# Autodesk Inventor assembly: kiteAssembly
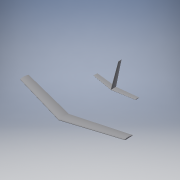
[picture p0: Inventor's stored thumbnail of the model, 180x180]
Saved by Autodesk Inventor 2019.3 (Build 233278000, 278)
## iProperties
Created: 2019-06-24
Part Number: kiteAssembly
Document SubType Name: Assembly
Designer: asiddiq2
Mass: 945352 g
Surface Area: 240754 cm^2
Volume: 945352 cm^3
Density: 1 g/cm^3
Author: asiddiq2
## Documents named in this file (4)
- C:\Users\asiddiq2\Desktop\OCT_project\CAD_models\kiteAssembly.iam
- C:\Users\asiddiq2\Desktop\OCT_project\CAD_models\kite\camberedWing.ipt
- C:\Users\asiddiq2\Desktop\OCT_project\CAD_models\kite\symmetricHS.ipt
- C:\Users\asiddiq2\Desktop\OCT_project\CAD_models\kite\symmetricVS.ipt
## Components (3 placed, 3 different names)
1. camberedWing:1 — Flush:1, Flush:2, Flush:5, Flush:6, Flush:7, Flush:8
2. symmetricHS:1 — Flush:1, Flush:2, Flush:3, Mate:1, Flush:4, Flush:5
3. symmetricVS:1 — Flush:3, Mate:1, Flush:4
## Relationships (9: Flush 8, Mate 1)
- Flush:1: camberedWing:1 ↔ symmetricHS:1
- Flush:2: camberedWing:1 ↔ symmetricHS:1
- Flush:3: symmetricHS:1 ↔ symmetricVS:1
- Mate:1: symmetricHS:1 ↔ symmetricVS:1
- Flush:4: symmetricHS:1 ↔ symmetricVS:1
- Flush:5 (5000 mm): camberedWing:1 ↔ symmetricHS:1
- Flush:6: camberedWing:1
- Flush:7: camberedWing:1
- Flush:8: camberedWing:1
